# Autodesk Inventor assembly: Zlozenie_glowne
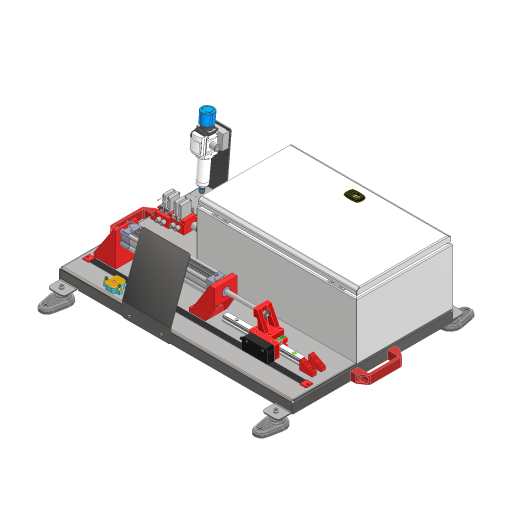
[picture p0: Inventor's stored thumbnail of the model, 512x512]
Saved by Autodesk Inventor 2024.3 (Build 283343000, 343)
## iProperties
Created: 2025-06-06
Part Number: Zlozenie_glowne
Document SubType Name: Assembly
Designer: PM
Author: PM
## Documents named in this file (45)
- C:\MPA - shortPath\magisterka\V3\Workspace\Zlozenie_glowne.iam
- C:\MPA - shortPath\magisterka\V3\Workspace\Stół.iam
- C:\MPA - shortPath\magisterka\V3\Workspace\Zakupowe\hiwin\HGH20CA1R250Z0H_FILE_1\HGH20CA1R250Z0H_FILE_1\HGH20CA1R250Z0H_FILE_1.iam
- C:\MPA - shortPath\magisterka\V3\Workspace\Part1.ipt
- C:\MPA - shortPath\magisterka\V3\Workspace\Zakupowe\silownik_metlawork\AIS2024\1213320200CP-0-0-0--(200_00).iam
- C:\MPA - shortPath\magisterka\V3\Workspace\cc\en-US\DIN 934\DIN 934 - M10 x 1,25.ipt
- C:\MPA - shortPath\magisterka\V3\Workspace\Part6.ipt
- C:\MPA - shortPath\magisterka\V3\Workspace\cc\en-US\DIN 125-1  A\DIN 125 - A 6,4.ipt
- C:\MPA - shortPath\magisterka\V3\Workspace\cc\en-US\DIN 912\DIN 912 - M6 x 1 x 20 x 17,5.ipt
- C:\MPA - shortPath\magisterka\V3\Workspace\cc\en-US\DIN 912\DIN 912 - M6 x 1 x 25 x 22,5.ipt
- C:\MPA - shortPath\magisterka\V3\Workspace\cc\en-US\DIN 934\DIN 934 - M6 x 1.ipt
- C:\MPA - shortPath\magisterka\V3\Workspace\fin.ipt
- C:\MPA - shortPath\magisterka\V3\Workspace\cc\en-US\DIN 912\DIN 912 - M5 x 0,8 x 20 x 18.ipt
- C:\MPA - shortPath\magisterka\V3\Workspace\cc\en-US\DIN 125-1  A\DIN 125 - A 5,3.ipt
- C:\MPA - shortPath\magisterka\V3\Workspace\cc\en-US\DIN 934\DIN 934 - M5 x 0,8.ipt
- C:\MPA - shortPath\magisterka\V3\Workspace\Zakupowe\lika\LIKA SMAX-MB-PRG-L2\LIKA SMAX-MB-PRG-L2\LIKA SMAX-MB-PRG-L2.ipt
- C:\MPA - shortPath\magisterka\V3\Workspace\Zakupowe\lika\MTAZ-500-50-1.ipt
- C:\MPA - shortPath\magisterka\V3\Workspace\Zakupowe\lika\LIKA LKM-1439.ipt
- C:\MPA - shortPath\magisterka\V3\Workspace\cc\en-US\ISO 10642(2)\ISO 10642  - M3  x  10.ipt
- C:\MPA - shortPath\magisterka\V3\Workspace\cc\en-US\DIN 125-1  A\DIN 125 - A 3,2.ipt
- C:\MPA - shortPath\magisterka\V3\Workspace\cc\en-US\DIN 934\DIN 934 - M3 x 0,5.ipt
- C:\MPA - shortPath\magisterka\V3\Workspace\blokada_hiwin.ipt
- C:\MPA - shortPath\magisterka\V3\Workspace\cc\en-US\DIN 912\DIN 912 - M4 x 0,7 x 16 x 14,25.ipt
- C:\MPA - shortPath\magisterka\V3\Workspace\cc\en-US\DIN 125-1  A\DIN 125 - A 4,3.ipt
- C:\MPA - shortPath\magisterka\V3\Workspace\cc\en-US\DIN 934\DIN 934 - M4 x 0,7.ipt
- C:\MPA - shortPath\magisterka\V3\Workspace\Zlozenie_smc.iam
- C:\MPA - shortPath\magisterka\V3\Workspace\Zakupowe\FESTO\MS4-EM1FR-14-D6-E-P-M-AG-MPA-WPE-B\8098374 MS4-EM1FR-1_4-D6-E-P-M-AG-MPA-WPE-B.iam
- C:\MPA - shortPath\magisterka\V3\Workspace\Zakupowe\smc\KQ2S06-01AS_(A) Brass.ipt
- C:\MPA - shortPath\magisterka\V3\Workspace\Part15.ipt
- C:\MPA - shortPath\magisterka\V3\Workspace\cc\en-US\DIN 912\DIN 912 - M4 x 0,7 x 30 x 20.ipt
- C:\MPA - shortPath\magisterka\V3\Workspace\Zakupowe\schneider\NSYS3D5320P_3D-Simplified\NSYS3D5320P_3D-Simplified\NSYS3D5320P_3D-Simplified.iam
- C:\MPA - shortPath\magisterka\V3\Workspace\Uchwyt_ZPP.ipt
- C:\MPA - shortPath\magisterka\V3\Workspace\cc\en-US\Copy of DIN 912 - replaced by DIN EN ISO 4762\Copy of DIN 912 - M5 x 0,8 x 16 x 14.ipt
- C:\MPA - shortPath\magisterka\V3\Workspace\cc\en-US\Copy of DIN 912 - replaced by DIN EN ISO 4762\Copy of DIN 912 - M4 x 0,7 x 20 x 18,25.ipt
- C:\MPA - shortPath\magisterka\V3\Workspace\Zakupowe\elesa\M_443_140-6-CH-C6\M_443_140-6-CH-C6\M_443_140-6-CH-C6.ipt
- C:\MPA - shortPath\magisterka\V3\Workspace\cc\en-US\Copy of DIN 912 - replaced by DIN EN ISO 4762\Copy of DIN 912 - M6 x 1 x 20 x 17,5.ipt
- C:\MPA - shortPath\magisterka\V3\Workspace\cc\en-US\DIN 9021\DIN 9021 - 8,4.ipt
- C:\MPA - shortPath\magisterka\V3\Workspace\cc\en-US\DIN 125-1  A\DIN 125 - A 8,4.ipt
- C:\MPA - shortPath\magisterka\V3\Workspace\cc\en-US\Copy of DIN 912 - replaced by DIN EN ISO 4762\Copy of DIN 912 - M8 x 1,25 x 20 x 16,875.ipt
- C:\MPA - shortPath\magisterka\V3\Workspace\cc\en-US\DIN 934\DIN 934 - M8 x 1,25.ipt
- C:\MPA - shortPath\magisterka\V3\Workspace\Arduino_zlozenie.iam
- C:\MPA - shortPath\magisterka\V3\Workspace\MontazWszafie\Uchwyt_konwerter.iam
- C:\MPA - shortPath\magisterka\V3\Workspace\cc\en-US\Copy of DIN 912 - replaced by DIN EN ISO 4762\Copy of DIN 912 - M4 x 0,7 x 12 x 10,25.ipt
- C:\MPA - shortPath\magisterka\V3\Workspace\PrzyciskSTOP.iam
- C:\MPA - shortPath\magisterka\V3\Workspace\cc\en-US\Copy of DIN 912 - replaced by DIN EN ISO 4762\Copy of DIN 912 - M4 x 0,7 x 25 x 23,25.ipt
## Components (187 placed, 44 different names)
1. Stół:1 [sub-assembly] — Flush:1, Flush:2, Flush:3, Insert:1, Mate:1, Flush:4, Mate:12, Mate:14, Mate:16, Mate:18, Mate:20, Mate:21, Mate:22, Mate:23, Mate:24, Mate:25, Mate:26, Mate:27, Mate:29, Mate:31, Mate:33, Mate:35, Mate:37, Mate:38, Mate:39, Mate:40, Mate:41, Mate:42, Mate:43, Mate:44, Mate:46, Flush:7, Mate:54, Mate:57, Mate:59, Mate:62, Mate:63, Mate:65, Mate:67, Mate:69, Mate:71, Mate:72, Mate:73, Mate:74, Mate:75, Mate:76, Mate:77, Mate:78, Mate:79, Flush:12, Mate:92, Mate:94, Mate:96, Mate:98, Mate:107, Flush:13, Flush:14, Flush:15, Mate:109, Flush:16, Flush:17, Mate:119, Mate:121, Mate:123, Mate:125, Mate:131, Mate:133, Mate:134, Flush:18, Flush:19, Mate:140, Mate:142, Flush:20, Mate:143, Mate:144, Mate:145, Mate:146, Mate:148, Mate:150, Mate:151, Mate:152, Mate:153, Mate:154, Mate:156, Mate:158, Mate:159, Mate:160, Mate:161, Mate:162, Mate:164, Mate:166, Mate:168, Mate:170, Mate:171, Mate:172, Mate:173, Mate:174, Mate:175, Mate:176, Mate:177, Mate:196, Flush:24
2. HGH20CA1R250Z0H_FILE_1:1 [sub-assembly] — Insert:1, Mate:1, Insert:2, Mate:2, Mate:30, Mate:32, Mate:34, Mate:36, Mate:58, Flush:8, Mate:60
3. Part1:1 — Insert:2, Mate:2, Insert:3, Insert:4, Angle:1, Insert:22, Mate:45, Mate:61, Mate:99, Mate:101, Mate:103, Mate:104, Mate:105, Mate:106
4. 1213320200CP-0-0-0--(200_00):1 [sub-assembly] — Insert:3, Angle:1, Insert:5, Mate:3, Flush:4, Insert:31, Insert:32, Insert:33
5. Part6:1 — Insert:5, Mate:3, Mate:4, Mate:5, Mate:6, Mate:7, Mate:8, Mate:9, Mate:10, Mate:11, Mate:13, Mate:15, Mate:17, Mate:19
6. fin:1 — Mate:134, Flush:18, Flush:19, Mate:135, Mate:136, Mate:137, Mate:138, Mate:139, Mate:141
7. LIKA SMAX-MB-PRG-L2:1 — Insert:22, Mate:45, Flush:5, Mate:100, Mate:102
8. MTAZ-500-50-1:1 — Mate:46, Flush:5, Mate:47, Mate:48, Mate:49, Mate:50, Mate:51
9. LIKA LKM-1439:1 — Mate:47, Mate:48, Mate:49, Flush:6, Flush:7, Mate:52, Mate:53
10. LIKA LKM-1439:2 — Flush:6, Mate:50, Mate:51, Mate:55, Mate:56
11. blokada_hiwin:1 — Mate:58, Mate:59, Flush:8, Mate:60, Flush:9, Mate:64, Mate:66, Mate:68, Mate:70
12. blokada_hiwin:2 — Mate:61, Flush:9, Mate:62
13. Zlozenie_smc:1 [sub-assembly] — Mate:79, Flush:12, Flush:15, Mate:126, Mate:127, Mate:128, Mate:129, Mate:130, Mate:132, Flush:23
14. 8098374 MS4-EM1FR-1_4-D6-E-P-M-AG-MPA-WPE-B:1 [sub-assembly] — Insert:42, Mate:108
15. KQ2S06-01AS_(A) Brass:1 — Insert:32
16. KQ2S06-01AS_(A) Brass:2 — Insert:31
17. Part15:1 — Insert:33, Mate:83, Mate:84, Mate:85, Mate:86, Mate:87, Mate:88, Mate:89, Mate:90, Mate:91, Mate:93, Mate:95, Mate:97
18. NSYS3D5320P_3D-Simplified:1 [sub-assembly] — Mate:107, Flush:13, Flush:14, Mate:163, Mate:165, Mate:167, Mate:169
19. Uchwyt_ZPP:1 — Insert:42, Mate:108, Mate:109, Flush:16, Flush:17, Mate:110, Mate:111, Mate:112, Mate:113, Mate:114, Mate:115, Mate:116, Mate:117, Mate:118, Mate:120, Mate:122, Mate:124, Mate:178, Mate:179, Mate:180, Mate:181, Mate:182, Mate:183, Mate:184, Mate:185, Mate:186, Mate:187, Mate:188, Mate:189, Mate:190, Mate:191, Mate:192, Mate:193
20. M_443_140-6-CH-C6:1 — Flush:20, Flush:21, Mate:143, Flush:22, Mate:145, Mate:155, Mate:157
21. M_443_140-6-CH-C6:2 — Flush:21, Mate:144, Flush:22, Mate:147, Mate:149
22. Arduino_zlozenie:1 [sub-assembly]
23. Uchwyt_konwerter:1 [sub-assembly]
24. PrzyciskSTOP:1 [sub-assembly] — Mate:196, Flush:24, Mate:197, Mate:198, Mate:199, Mate:200
25. DIN 125-1 A A 4,3:9 — Mate:178, Mate:179, Insert:79
26. Copy of DIN 912 - replaced by DIN EN ISO 4762 M4 x 12:1 — Insert:79
27. DIN 125-1 A A 4,3:10 — Mate:186, Mate:187, Insert:83
28. DIN 934 - replaced by DIN EN 24032/28673/28674 M4:9 — Insert:83
29. DIN 125-1 A A 4,3:11 — Mate:180, Mate:181, Insert:80
30. DIN 125-1 A A 4,3:12 — Mate:182, Mate:183, Insert:81
31. DIN 125-1 A A 4,3:13 — Mate:184, Mate:185, Insert:82
32. Copy of DIN 912 - replaced by DIN EN ISO 4762 M4 x 12:2 — Insert:80
33. Copy of DIN 912 - replaced by DIN EN ISO 4762 M4 x 12:3 — Insert:81
34. Copy of DIN 912 - replaced by DIN EN ISO 4762 M4 x 12:4 — Insert:82
35. DIN 125-1 A A 4,3:14 — Mate:188, Mate:189, Insert:84
36. DIN 125-1 A A 4,3:15 — Mate:190, Mate:191, Insert:85
37. DIN 125-1 A A 4,3:16 — Mate:192, Mate:193, Insert:86
38. DIN 934 - replaced by DIN EN 24032/28673/28674 M4:10 — Insert:84
39. DIN 934 - replaced by DIN EN 24032/28673/28674 M4:11 — Insert:85
40. DIN 934 - replaced by DIN EN 24032/28673/28674 M4:12 — Insert:86
41. DIN 125-1 A A 4,3:17 — Mate:197, Mate:198, Insert:87
42. Copy of DIN 912 - replaced by DIN EN ISO 4762 M4 x 25:1 — Insert:87
43. DIN 125-1 A A 4,3:18 — Mate:199, Mate:200, Insert:88
44. Copy of DIN 912 - replaced by DIN EN ISO 4762 M4 x 25:2 — Insert:88
45. DIN 9021 8,4:1 — Mate:162, Mate:163, Insert:63
46. DIN 125-1 A A 8,4:1 — Insert:63, Insert:67
47. Copy of DIN 912 - replaced by DIN EN ISO 4762 M8 x 20:1 — Insert:67
48. DIN 125-1 A A 8,4:2 — Mate:170, Mate:171, Insert:71
49. DIN 9021 8,4:2 — Insert:71, Insert:75
50. DIN 934 - replaced by DIN EN 24032/28673/28674 M8:1 — Insert:75
51. DIN 9021 8,4:3 — Mate:164, Mate:165, Insert:64
52. DIN 9021 8,4:4 — Mate:166, Mate:167, Insert:65
53. DIN 9021 8,4:5 — Mate:168, Mate:169, Insert:66
54. DIN 125-1 A A 8,4:3 — Insert:64, Insert:68
55. DIN 125-1 A A 8,4:4 — Insert:65, Insert:69
56. DIN 125-1 A A 8,4:5 — Insert:66, Insert:70
57. Copy of DIN 912 - replaced by DIN EN ISO 4762 M8 x 20:2 — Insert:68
58. Copy of DIN 912 - replaced by DIN EN ISO 4762 M8 x 20:3 — Insert:69
59. Copy of DIN 912 - replaced by DIN EN ISO 4762 M8 x 20:4 — Insert:70
60. DIN 125-1 A A 8,4:6 — Mate:172, Mate:173, Insert:72
61. DIN 125-1 A A 8,4:7 — Mate:174, Mate:175, Insert:73
62. DIN 125-1 A A 8,4:8 — Mate:176, Mate:177, Insert:74
63. DIN 9021 8,4:6 — Insert:72, Insert:76
64. DIN 9021 8,4:7 — Insert:73, Insert:77
65. DIN 9021 8,4:8 — Insert:74, Insert:78
66. DIN 934 - replaced by DIN EN 24032/28673/28674 M8:2 — Insert:76
67. DIN 934 - replaced by DIN EN 24032/28673/28674 M8:3 — Insert:77
68. DIN 934 - replaced by DIN EN 24032/28673/28674 M8:4 — Insert:78
69. DIN 125-1 A A 5,3:5 — Mate:110, Mate:111, Insert:43
70. Copy of DIN 912 - replaced by DIN EN ISO 4762 M5 x 16:1 — Insert:43
71. DIN 125-1 A A 5,3:6 — Mate:118, Mate:119, Insert:47
72. DIN 934 - replaced by DIN EN 24032/28673/28674 M5:5 — Insert:47
73. DIN 125-1 A A 5,3:7 — Mate:112, Mate:113, Insert:44
74. DIN 125-1 A A 5,3:8 — Mate:114, Mate:115, Insert:45
75. DIN 125-1 A A 5,3:9 — Mate:116, Mate:117, Insert:46
76. Copy of DIN 912 - replaced by DIN EN ISO 4762 M5 x 16:2 — Insert:44
77. Copy of DIN 912 - replaced by DIN EN ISO 4762 M5 x 16:3 — Insert:45
78. Copy of DIN 912 - replaced by DIN EN ISO 4762 M5 x 16:4 — Insert:46
79. DIN 125-1 A A 5,3:10 — Mate:120, Mate:121, Insert:48
80. DIN 125-1 A A 5,3:11 — Mate:122, Mate:123, Insert:49
81. DIN 125-1 A A 5,3:12 — Mate:124, Mate:125, Insert:50
82. DIN 934 - replaced by DIN EN 24032/28673/28674 M5:6 — Insert:48
83. DIN 934 - replaced by DIN EN 24032/28673/28674 M5:7 — Insert:49
84. DIN 934 - replaced by DIN EN 24032/28673/28674 M5:8 — Insert:50
85. DIN 125-1 A A 4,3:5 — Mate:126, Mate:127, Insert:51
86. Copy of DIN 912 - replaced by DIN EN ISO 4762 M4 x 20:1 — Insert:51
87. DIN 125-1 A A 4,3:6 — Mate:130, Mate:131, Insert:53
88. DIN 934 - replaced by DIN EN 24032/28673/28674 M4:7 — Insert:53
89. DIN 125-1 A A 4,3:7 — Mate:128, Mate:129, Insert:52
90. Copy of DIN 912 - replaced by DIN EN ISO 4762 M4 x 20:2 — Insert:52
91. DIN 125-1 A A 4,3:8 — Mate:132, Mate:133, Insert:54
92. DIN 934 - replaced by DIN EN 24032/28673/28674 M4:8 — Insert:54
93. DIN 125-1 A A 5,3:13 — Mate:135, Mate:136, Insert:55
94. Copy of DIN 912 - replaced by DIN EN ISO 4762 M5 x 16:5 — Insert:55
95. DIN 125-1 A A 5,3:14 — Mate:139, Mate:140, Insert:57
96. DIN 934 - replaced by DIN EN 24032/28673/28674 M5:9 — Insert:57
97. DIN 125-1 A A 5,3:15 — Mate:137, Mate:138, Insert:56
98. Copy of DIN 912 - replaced by DIN EN ISO 4762 M5 x 16:6 — Insert:56
99. DIN 125-1 A A 5,3:16 — Mate:141, Mate:142, Insert:58
100. DIN 934 - replaced by DIN EN 24032/28673/28674 M5:10 — Insert:58
101. Copy of DIN 912 - replaced by DIN EN ISO 4762 M6 x 20:1 — Mate:146, Mate:147
102. DIN 125-1 A A 6,4:21 — Mate:150, Mate:151, Insert:59
103. DIN 934 - replaced by DIN EN 24032/28673/28674 M6:9 — Insert:59
104. Copy of DIN 912 - replaced by DIN EN ISO 4762 M6 x 20:2 — Mate:148, Mate:149
105. DIN 125-1 A A 6,4:22 — Mate:152, Mate:153, Insert:60
106. DIN 934 - replaced by DIN EN 24032/28673/28674 M6:10 — Insert:60
107. Copy of DIN 912 - replaced by DIN EN ISO 4762 M6 x 20:3 — Mate:154, Mate:155
108. DIN 125-1 A A 6,4:23 — Mate:158, Mate:159, Insert:61
109. DIN 934 - replaced by DIN EN 24032/28673/28674 M6:11 — Insert:61
110. Copy of DIN 912 - replaced by DIN EN ISO 4762 M6 x 20:4 — Mate:156, Mate:157
111. DIN 125-1 A A 6,4:24 — Mate:160, Mate:161, Insert:62
112. DIN 934 - replaced by DIN EN 24032/28673/28674 M6:12 — Insert:62
113. DIN 912 - replaced by DIN EN ISO 4762 M4 x 30:1 — Mate:99, Mate:100
114. DIN 934 - replaced by DIN EN 24032/28673/28674 M4:5 — Mate:103, Mate:104
115. DIN 912 - replaced by DIN EN ISO 4762 M4 x 30:2 — Mate:101, Mate:102
116. DIN 934 - replaced by DIN EN 24032/28673/28674 M4:6 — Mate:105, Mate:106
117. DIN 125-1 A A 6,4:13 — Mate:83, Mate:84, Insert:34
118. DIN 912 - replaced by DIN EN ISO 4762 M6 x 25:5 — Insert:34
119. DIN 125-1 A A 6,4:14 — Mate:91, Mate:92, Insert:38
120. DIN 934 - replaced by DIN EN 24032/28673/28674 M6:5 — Insert:38
121. DIN 125-1 A A 6,4:15 — Mate:85, Mate:86, Insert:35
122. DIN 125-1 A A 6,4:16 — Mate:87, Mate:88, Insert:36
123. DIN 125-1 A A 6,4:17 — Mate:89, Mate:90, Insert:37
124. DIN 912 - replaced by DIN EN ISO 4762 M6 x 25:6 — Insert:35
125. DIN 912 - replaced by DIN EN ISO 4762 M6 x 25:7 — Insert:36
126. DIN 912 - replaced by DIN EN ISO 4762 M6 x 25:8 — Insert:37
127. DIN 125-1 A A 6,4:18 — Mate:93, Mate:94, Insert:39
128. DIN 125-1 A A 6,4:19 — Mate:95, Mate:96, Insert:40
129. DIN 125-1 A A 6,4:20 — Mate:97, Mate:98, Insert:41
130. DIN 934 - replaced by DIN EN 24032/28673/28674 M6:6 — Insert:39
131. DIN 934 - replaced by DIN EN 24032/28673/28674 M6:7 — Insert:40
132. DIN 934 - replaced by DIN EN 24032/28673/28674 M6:8 — Insert:41
133. DIN 912 - replaced by DIN EN ISO 4762 M4 x 16:1 — Mate:63, Mate:64
134. DIN 125-1 A A 4,3:1 — Mate:71, Mate:72, Insert:25
135. DIN 934 - replaced by DIN EN 24032/28673/28674 M4:1 — Insert:25
136. DIN 912 - replaced by DIN EN ISO 4762 M4 x 16:2 — Mate:65, Mate:66
137. DIN 912 - replaced by DIN EN ISO 4762 M4 x 16:3 — Mate:67, Mate:68
138. DIN 912 - replaced by DIN EN ISO 4762 M4 x 16:4 — Mate:69, Mate:70
139. DIN 125-1 A A 4,3:2 — Mate:73, Mate:74, Insert:26
140. DIN 125-1 A A 4,3:3 — Mate:75, Mate:76, Insert:27
141. DIN 125-1 A A 4,3:4 — Mate:77, Mate:78, Insert:28
142. DIN 934 - replaced by DIN EN 24032/28673/28674 M4:2 — Insert:26
143. DIN 934 - replaced by DIN EN 24032/28673/28674 M4:3 — Insert:27
144. DIN 934 - replaced by DIN EN 24032/28673/28674 M4:4 — Insert:28
145. DIN EN ISO 10642 M3  x  10:1 — Mate:52
146. DIN 125-1 A A 3,2:1 — Mate:53, Mate:54, Insert:23
147. DIN 934 - replaced by DIN EN 24032/28673/28674 M3:1 — Insert:23
148. DIN EN ISO 10642 M3  x  10:2 — Mate:55
149. DIN 125-1 A A 3,2:2 — Mate:56, Mate:57, Insert:24
150. DIN 934 - replaced by DIN EN 24032/28673/28674 M3:2 — Insert:24
151. DIN 912 - replaced by DIN EN ISO 4762 M5 x 20:1 — Mate:29, Mate:30
152. DIN 125-1 A A 5,3:1 — Mate:37, Mate:38, Insert:18
153. DIN 934 - replaced by DIN EN 24032/28673/28674 M5:1 — Insert:18
154. DIN 912 - replaced by DIN EN ISO 4762 M5 x 20:2 — Mate:31, Mate:32
155. DIN 912 - replaced by DIN EN ISO 4762 M5 x 20:3 — Mate:33, Mate:34
156. DIN 912 - replaced by DIN EN ISO 4762 M5 x 20:4 — Mate:35, Mate:36
157. DIN 125-1 A A 5,3:2 — Mate:39, Mate:40, Insert:19
158. DIN 125-1 A A 5,3:3 — Mate:41, Mate:42, Insert:20
159. DIN 125-1 A A 5,3:4 — Mate:43, Mate:44, Insert:21
160. DIN 934 - replaced by DIN EN 24032/28673/28674 M5:2 — Insert:19
161. DIN 934 - replaced by DIN EN 24032/28673/28674 M5:3 — Insert:20
162. DIN 934 - replaced by DIN EN 24032/28673/28674 M5:4 — Insert:21
163. DIN 125-1 A A 6,4:1 — Mate:4, Mate:5, Insert:6
164. DIN 912 - replaced by DIN EN ISO 4762 M6 x 20:1 — Insert:6
165. DIN 125-1 A A 6,4:2 — Mate:6, Mate:7, Insert:7
166. DIN 125-1 A A 6,4:3 — Mate:8, Mate:9, Insert:8
167. DIN 125-1 A A 6,4:4 — Mate:10, Mate:11, Insert:9
168. DIN 912 - replaced by DIN EN ISO 4762 M6 x 20:2 — Insert:7
169. DIN 912 - replaced by DIN EN ISO 4762 M6 x 20:3 — Insert:8
170. DIN 912 - replaced by DIN EN ISO 4762 M6 x 20:4 — Insert:9
171. DIN 125-1 A A 6,4:5 — Mate:12, Mate:13, Insert:10
172. DIN 912 - replaced by DIN EN ISO 4762 M6 x 25:1 — Insert:10
173. DIN 125-1 A A 6,4:6 — Mate:20, Mate:21, Insert:14
174. DIN 934 - replaced by DIN EN 24032/28673/28674 M6:1 — Insert:14
175. DIN 125-1 A A 6,4:7 — Mate:14, Mate:15, Insert:11
176. DIN 125-1 A A 6,4:8 — Mate:16, Mate:17, Insert:12
177. DIN 125-1 A A 6,4:9 — Mate:18, Mate:19, Insert:13
178. DIN 912 - replaced by DIN EN ISO 4762 M6 x 25:2 — Insert:11
179. DIN 912 - replaced by DIN EN ISO 4762 M6 x 25:3 — Insert:12
180. DIN 912 - replaced by DIN EN ISO 4762 M6 x 25:4 — Insert:13
181. DIN 125-1 A A 6,4:10 — Mate:22, Mate:23, Insert:15
182. DIN 125-1 A A 6,4:11 — Mate:24, Mate:25, Insert:16
183. DIN 125-1 A A 6,4:12 — Mate:26, Mate:27, Insert:17
184. DIN 934 - replaced by DIN EN 24032/28673/28674 M6:2 — Insert:15
185. DIN 934 - replaced by DIN EN 24032/28673/28674 M6:3 — Insert:16
186. DIN 934 - replaced by DIN EN 24032/28673/28674 M6:4 — Insert:17
187. DIN 934 - replaced by DIN EN 24032/28673/28674 M10 x 1,25:1 — Insert:4
## Relationships (304: Mate 195, Insert 86, Flush 22, Angle 1)
- Flush:1: Stół:1
- Flush:2: Stół:1
- Flush:3: Stół:1
- Insert:1: Stół:1 ↔ HGH20CA1R250Z0H_FILE_1:1
- Mate:1: Stół:1 ↔ HGH20CA1R250Z0H_FILE_1:1
- Insert:2: HGH20CA1R250Z0H_FILE_1:1 ↔ Part1:1
- Mate:2: HGH20CA1R250Z0H_FILE_1:1 ↔ Part1:1
- Insert:3: Part1:1 ↔ 1213320200CP-0-0-0--(200_00):1
- Insert:4: Part1:1 ↔ DIN 934 - replaced by DIN EN 24032/28673/28674 M10 x 1,25:1
- Angle:1 (0 deg): Part1:1 ↔ 1213320200CP-0-0-0--(200_00):1
- Insert:5: 1213320200CP-0-0-0--(200_00):1 ↔ Part6:1
- Mate:3: 1213320200CP-0-0-0--(200_00):1 ↔ Part6:1
- Flush:4 (91.5 mm): Stół:1 ↔ 1213320200CP-0-0-0--(200_00):1
- Mate:4: Part6:1 ↔ DIN 125-1 A A 6,4:1
- Mate:5: Part6:1 ↔ DIN 125-1 A A 6,4:1
- Mate:6: Part6:1 ↔ DIN 125-1 A A 6,4:2
- Mate:7: Part6:1 ↔ DIN 125-1 A A 6,4:2
- Mate:8: Part6:1 ↔ DIN 125-1 A A 6,4:3
- Mate:9: Part6:1 ↔ DIN 125-1 A A 6,4:3
- Mate:10: Part6:1 ↔ DIN 125-1 A A 6,4:4
- Mate:11: Part6:1 ↔ DIN 125-1 A A 6,4:4
- Insert:6: DIN 125-1 A A 6,4:1 ↔ DIN 912 - replaced by DIN EN ISO 4762 M6 x 20:1
- Insert:7: DIN 125-1 A A 6,4:2 ↔ DIN 912 - replaced by DIN EN ISO 4762 M6 x 20:2
- Insert:8: DIN 125-1 A A 6,4:3 ↔ DIN 912 - replaced by DIN EN ISO 4762 M6 x 20:3
- Insert:9: DIN 125-1 A A 6,4:4 ↔ DIN 912 - replaced by DIN EN ISO 4762 M6 x 20:4
- Mate:12: Stół:1 ↔ DIN 125-1 A A 6,4:5
- Mate:13: Part6:1 ↔ DIN 125-1 A A 6,4:5
- Mate:14: Stół:1 ↔ DIN 125-1 A A 6,4:7
- Mate:15: Part6:1 ↔ DIN 125-1 A A 6,4:7
- Mate:16: Stół:1 ↔ DIN 125-1 A A 6,4:8
- Mate:17: Part6:1 ↔ DIN 125-1 A A 6,4:8
- Mate:18: Stół:1 ↔ DIN 125-1 A A 6,4:9
- Mate:19: Part6:1 ↔ DIN 125-1 A A 6,4:9
- Insert:10: DIN 125-1 A A 6,4:5 ↔ DIN 912 - replaced by DIN EN ISO 4762 M6 x 25:1
- Insert:11: DIN 125-1 A A 6,4:7 ↔ DIN 912 - replaced by DIN EN ISO 4762 M6 x 25:2
- Insert:12: DIN 125-1 A A 6,4:8 ↔ DIN 912 - replaced by DIN EN ISO 4762 M6 x 25:3
- Insert:13: DIN 125-1 A A 6,4:9 ↔ DIN 912 - replaced by DIN EN ISO 4762 M6 x 25:4
- Mate:20: Stół:1 ↔ DIN 125-1 A A 6,4:6
- Mate:21: Stół:1 ↔ DIN 125-1 A A 6,4:6
- Mate:22: Stół:1 ↔ DIN 125-1 A A 6,4:10
- Mate:23: Stół:1 ↔ DIN 125-1 A A 6,4:10
- Mate:24: Stół:1 ↔ DIN 125-1 A A 6,4:11
- Mate:25: Stół:1 ↔ DIN 125-1 A A 6,4:11
- Mate:26: Stół:1 ↔ DIN 125-1 A A 6,4:12
- Mate:27: Stół:1 ↔ DIN 125-1 A A 6,4:12
- Insert:14: DIN 125-1 A A 6,4:6 ↔ DIN 934 - replaced by DIN EN 24032/28673/28674 M6:1
- Insert:15: DIN 125-1 A A 6,4:10 ↔ DIN 934 - replaced by DIN EN 24032/28673/28674 M6:2
- Insert:16: DIN 125-1 A A 6,4:11 ↔ DIN 934 - replaced by DIN EN 24032/28673/28674 M6:3
- Insert:17: DIN 125-1 A A 6,4:12 ↔ DIN 934 - replaced by DIN EN 24032/28673/28674 M6:4
- Mate:29: Stół:1 ↔ DIN 912 - replaced by DIN EN ISO 4762 M5 x 20:1
- Mate:30: HGH20CA1R250Z0H_FILE_1:1 ↔ DIN 912 - replaced by DIN EN ISO 4762 M5 x 20:1
- Mate:31: Stół:1 ↔ DIN 912 - replaced by DIN EN ISO 4762 M5 x 20:2
- Mate:32: HGH20CA1R250Z0H_FILE_1:1 ↔ DIN 912 - replaced by DIN EN ISO 4762 M5 x 20:2
- Mate:33: Stół:1 ↔ DIN 912 - replaced by DIN EN ISO 4762 M5 x 20:3
- Mate:34: HGH20CA1R250Z0H_FILE_1:1 ↔ DIN 912 - replaced by DIN EN ISO 4762 M5 x 20:3
- Mate:35: Stół:1 ↔ DIN 912 - replaced by DIN EN ISO 4762 M5 x 20:4
- Mate:36: HGH20CA1R250Z0H_FILE_1:1 ↔ DIN 912 - replaced by DIN EN ISO 4762 M5 x 20:4
- Mate:37: Stół:1 ↔ DIN 125-1 A A 5,3:1
- Mate:38: Stół:1 ↔ DIN 125-1 A A 5,3:1
- Mate:39: Stół:1 ↔ DIN 125-1 A A 5,3:2
- Mate:40: Stół:1 ↔ DIN 125-1 A A 5,3:2
- Mate:41: Stół:1 ↔ DIN 125-1 A A 5,3:3
- Mate:42: Stół:1 ↔ DIN 125-1 A A 5,3:3
- Mate:43: Stół:1 ↔ DIN 125-1 A A 5,3:4
- Mate:44: Stół:1 ↔ DIN 125-1 A A 5,3:4
- Insert:18: DIN 125-1 A A 5,3:1 ↔ DIN 934 - replaced by DIN EN 24032/28673/28674 M5:1
- Insert:19: DIN 125-1 A A 5,3:2 ↔ DIN 934 - replaced by DIN EN 24032/28673/28674 M5:2
- Insert:20: DIN 125-1 A A 5,3:3 ↔ DIN 934 - replaced by DIN EN 24032/28673/28674 M5:3
- Insert:21: DIN 125-1 A A 5,3:4 ↔ DIN 934 - replaced by DIN EN 24032/28673/28674 M5:4
- Insert:22: Part1:1 ↔ LIKA SMAX-MB-PRG-L2:1
- Mate:45: Part1:1 ↔ LIKA SMAX-MB-PRG-L2:1
- Mate:46: Stół:1 ↔ MTAZ-500-50-1:1
- Flush:5 (1 mm): LIKA SMAX-MB-PRG-L2:1 ↔ MTAZ-500-50-1:1
- Mate:47: MTAZ-500-50-1:1 ↔ LIKA LKM-1439:1
- Mate:48: MTAZ-500-50-1:1 ↔ LIKA LKM-1439:1
- Mate:49 (0.1 mm): MTAZ-500-50-1:1 ↔ LIKA LKM-1439:1
- Flush:6: LIKA LKM-1439:1 ↔ LIKA LKM-1439:2
- Mate:50: MTAZ-500-50-1:1 ↔ LIKA LKM-1439:2
- Mate:51: MTAZ-500-50-1:1 ↔ LIKA LKM-1439:2
- Flush:7 (15 mm): Stół:1 ↔ LIKA LKM-1439:1
- Mate:52: LIKA LKM-1439:1 ↔ DIN EN ISO 10642 M3  x  10:1
- Mate:53: LIKA LKM-1439:1 ↔ DIN 125-1 A A 3,2:1
- Mate:54: Stół:1 ↔ DIN 125-1 A A 3,2:1
- Insert:23: DIN 125-1 A A 3,2:1 ↔ DIN 934 - replaced by DIN EN 24032/28673/28674 M3:1
- Mate:55: LIKA LKM-1439:2 ↔ DIN EN ISO 10642 M3  x  10:2
- Mate:56: LIKA LKM-1439:2 ↔ DIN 125-1 A A 3,2:2
- Mate:57: Stół:1 ↔ DIN 125-1 A A 3,2:2
- Insert:24: DIN 125-1 A A 3,2:2 ↔ DIN 934 - replaced by DIN EN 24032/28673/28674 M3:2
- Mate:58 (1 mm): HGH20CA1R250Z0H_FILE_1:1 ↔ blokada_hiwin:1
- Mate:59: Stół:1 ↔ blokada_hiwin:1
- Flush:8: HGH20CA1R250Z0H_FILE_1:1 ↔ blokada_hiwin:1
- Mate:60: HGH20CA1R250Z0H_FILE_1:1 ↔ blokada_hiwin:1
- Mate:61 (2 mm): Part1:1 ↔ blokada_hiwin:2
- Flush:9: blokada_hiwin:1 ↔ blokada_hiwin:2
- Mate:62: Stół:1 ↔ blokada_hiwin:2
- Mate:63: Stół:1 ↔ DIN 912 - replaced by DIN EN ISO 4762 M4 x 16:1
- Mate:64: blokada_hiwin:1 ↔ DIN 912 - replaced by DIN EN ISO 4762 M4 x 16:1
- Mate:65: Stół:1 ↔ DIN 912 - replaced by DIN EN ISO 4762 M4 x 16:2
- Mate:66: blokada_hiwin:1 ↔ DIN 912 - replaced by DIN EN ISO 4762 M4 x 16:2
- Mate:67: Stół:1 ↔ DIN 912 - replaced by DIN EN ISO 4762 M4 x 16:3
- Mate:68: blokada_hiwin:1 ↔ DIN 912 - replaced by DIN EN ISO 4762 M4 x 16:3
- Mate:69: Stół:1 ↔ DIN 912 - replaced by DIN EN ISO 4762 M4 x 16:4
- Mate:70: blokada_hiwin:1 ↔ DIN 912 - replaced by DIN EN ISO 4762 M4 x 16:4
- Mate:71: Stół:1 ↔ DIN 125-1 A A 4,3:1
- Mate:72: Stół:1 ↔ DIN 125-1 A A 4,3:1
- Mate:73: Stół:1 ↔ DIN 125-1 A A 4,3:2
- Mate:74: Stół:1 ↔ DIN 125-1 A A 4,3:2
- Mate:75: Stół:1 ↔ DIN 125-1 A A 4,3:3
- Mate:76: Stół:1 ↔ DIN 125-1 A A 4,3:3
- Mate:77: Stół:1 ↔ DIN 125-1 A A 4,3:4
- Mate:78: Stół:1 ↔ DIN 125-1 A A 4,3:4
- Insert:25: DIN 125-1 A A 4,3:1 ↔ DIN 934 - replaced by DIN EN 24032/28673/28674 M4:1
- Insert:26: DIN 125-1 A A 4,3:2 ↔ DIN 934 - replaced by DIN EN 24032/28673/28674 M4:2
- Insert:27: DIN 125-1 A A 4,3:3 ↔ DIN 934 - replaced by DIN EN 24032/28673/28674 M4:3
- Insert:28: DIN 125-1 A A 4,3:4 ↔ DIN 934 - replaced by DIN EN 24032/28673/28674 M4:4
- Mate:79: Stół:1 ↔ Zlozenie_smc:1
- Flush:12 (179.1 mm): Stół:1 ↔ Zlozenie_smc:1
- Insert:31: 1213320200CP-0-0-0--(200_00):1 ↔ KQ2S06-01AS_(A) Brass:2
- Insert:32: 1213320200CP-0-0-0--(200_00):1 ↔ KQ2S06-01AS_(A) Brass:1
- Insert:33: 1213320200CP-0-0-0--(200_00):1 ↔ Part15:1
- Mate:83: Part15:1 ↔ DIN 125-1 A A 6,4:13
- Mate:84: Part15:1 ↔ DIN 125-1 A A 6,4:13
- Mate:85: Part15:1 ↔ DIN 125-1 A A 6,4:15
- Mate:86: Part15:1 ↔ DIN 125-1 A A 6,4:15
- Mate:87: Part15:1 ↔ DIN 125-1 A A 6,4:16
- Mate:88: Part15:1 ↔ DIN 125-1 A A 6,4:16
- Mate:89: Part15:1 ↔ DIN 125-1 A A 6,4:17
- Mate:90: Part15:1 ↔ DIN 125-1 A A 6,4:17
- Insert:34: DIN 125-1 A A 6,4:13 ↔ DIN 912 - replaced by DIN EN ISO 4762 M6 x 25:5
- Insert:35: DIN 125-1 A A 6,4:15 ↔ DIN 912 - replaced by DIN EN ISO 4762 M6 x 25:6
- Insert:36: DIN 125-1 A A 6,4:16 ↔ DIN 912 - replaced by DIN EN ISO 4762 M6 x 25:7
- Insert:37: DIN 125-1 A A 6,4:17 ↔ DIN 912 - replaced by DIN EN ISO 4762 M6 x 25:8
- Mate:91: Part15:1 ↔ DIN 125-1 A A 6,4:14
- Mate:92: Stół:1 ↔ DIN 125-1 A A 6,4:14
- Mate:93: Part15:1 ↔ DIN 125-1 A A 6,4:18
- Mate:94: Stół:1 ↔ DIN 125-1 A A 6,4:18
- Mate:95: Part15:1 ↔ DIN 125-1 A A 6,4:19
- Mate:96: Stół:1 ↔ DIN 125-1 A A 6,4:19
- Mate:97: Part15:1 ↔ DIN 125-1 A A 6,4:20
- Mate:98: Stół:1 ↔ DIN 125-1 A A 6,4:20
- Insert:38: DIN 125-1 A A 6,4:14 ↔ DIN 934 - replaced by DIN EN 24032/28673/28674 M6:5
- Insert:39: DIN 125-1 A A 6,4:18 ↔ DIN 934 - replaced by DIN EN 24032/28673/28674 M6:6
- Insert:40: DIN 125-1 A A 6,4:19 ↔ DIN 934 - replaced by DIN EN 24032/28673/28674 M6:7
- Insert:41: DIN 125-1 A A 6,4:20 ↔ DIN 934 - replaced by DIN EN 24032/28673/28674 M6:8
- Mate:99: Part1:1 ↔ DIN 912 - replaced by DIN EN ISO 4762 M4 x 30:1
- Mate:100: LIKA SMAX-MB-PRG-L2:1 ↔ DIN 912 - replaced by DIN EN ISO 4762 M4 x 30:1
- Mate:101: Part1:1 ↔ DIN 912 - replaced by DIN EN ISO 4762 M4 x 30:2
- Mate:102: LIKA SMAX-MB-PRG-L2:1 ↔ DIN 912 - replaced by DIN EN ISO 4762 M4 x 30:2
- Mate:103: Part1:1 ↔ DIN 934 - replaced by DIN EN 24032/28673/28674 M4:5
- Mate:104: Part1:1 ↔ DIN 934 - replaced by DIN EN 24032/28673/28674 M4:5
- Mate:105: Part1:1 ↔ DIN 934 - replaced by DIN EN 24032/28673/28674 M4:6
- Mate:106: Part1:1 ↔ DIN 934 - replaced by DIN EN 24032/28673/28674 M4:6
- Mate:107: Stół:1 ↔ NSYS3D5320P_3D-Simplified:1
- Flush:13: Stół:1 ↔ NSYS3D5320P_3D-Simplified:1
- Flush:14: Stół:1 ↔ NSYS3D5320P_3D-Simplified:1
- Flush:15 (12.5 mm): Stół:1 ↔ Zlozenie_smc:1
- Insert:42: 8098374 MS4-EM1FR-1_4-D6-E-P-M-AG-MPA-WPE-B:1 ↔ Uchwyt_ZPP:1
- Mate:108: 8098374 MS4-EM1FR-1_4-D6-E-P-M-AG-MPA-WPE-B:1 ↔ Uchwyt_ZPP:1
- Mate:109: Stół:1 ↔ Uchwyt_ZPP:1
- Flush:16 (6 mm): Stół:1 ↔ Uchwyt_ZPP:1
- Flush:17 (6 mm): Stół:1 ↔ Uchwyt_ZPP:1
- Mate:110: Uchwyt_ZPP:1 ↔ DIN 125-1 A A 5,3:5
- Mate:111: Uchwyt_ZPP:1 ↔ DIN 125-1 A A 5,3:5
- Mate:112: Uchwyt_ZPP:1 ↔ DIN 125-1 A A 5,3:7
- Mate:113: Uchwyt_ZPP:1 ↔ DIN 125-1 A A 5,3:7
- Mate:114: Uchwyt_ZPP:1 ↔ DIN 125-1 A A 5,3:8
- Mate:115: Uchwyt_ZPP:1 ↔ DIN 125-1 A A 5,3:8
- Mate:116: Uchwyt_ZPP:1 ↔ DIN 125-1 A A 5,3:9
- Mate:117: Uchwyt_ZPP:1 ↔ DIN 125-1 A A 5,3:9
- Insert:43: DIN 125-1 A A 5,3:5 ↔ Copy of DIN 912 - replaced by DIN EN ISO 4762 M5 x 16:1
- Insert:44: DIN 125-1 A A 5,3:7 ↔ Copy of DIN 912 - replaced by DIN EN ISO 4762 M5 x 16:2
- Insert:45: DIN 125-1 A A 5,3:8 ↔ Copy of DIN 912 - replaced by DIN EN ISO 4762 M5 x 16:3
- Insert:46: DIN 125-1 A A 5,3:9 ↔ Copy of DIN 912 - replaced by DIN EN ISO 4762 M5 x 16:4
- Mate:118: Uchwyt_ZPP:1 ↔ DIN 125-1 A A 5,3:6
- Mate:119: Stół:1 ↔ DIN 125-1 A A 5,3:6
- Mate:120: Uchwyt_ZPP:1 ↔ DIN 125-1 A A 5,3:10
- Mate:121: Stół:1 ↔ DIN 125-1 A A 5,3:10
- Mate:122: Uchwyt_ZPP:1 ↔ DIN 125-1 A A 5,3:11
- Mate:123: Stół:1 ↔ DIN 125-1 A A 5,3:11
- Mate:124: Uchwyt_ZPP:1 ↔ DIN 125-1 A A 5,3:12
- Mate:125: Stół:1 ↔ DIN 125-1 A A 5,3:12
- Insert:47: DIN 125-1 A A 5,3:6 ↔ DIN 934 - replaced by DIN EN 24032/28673/28674 M5:5
- Insert:48: DIN 125-1 A A 5,3:10 ↔ DIN 934 - replaced by DIN EN 24032/28673/28674 M5:6
- Insert:49: DIN 125-1 A A 5,3:11 ↔ DIN 934 - replaced by DIN EN 24032/28673/28674 M5:7
- Insert:50: DIN 125-1 A A 5,3:12 ↔ DIN 934 - replaced by DIN EN 24032/28673/28674 M5:8
- Mate:126: Zlozenie_smc:1 ↔ DIN 125-1 A A 4,3:5
- Mate:127: Zlozenie_smc:1 ↔ DIN 125-1 A A 4,3:5
- Mate:128: Zlozenie_smc:1 ↔ DIN 125-1 A A 4,3:7
- Mate:129: Zlozenie_smc:1 ↔ DIN 125-1 A A 4,3:7
- Insert:51: DIN 125-1 A A 4,3:5 ↔ Copy of DIN 912 - replaced by DIN EN ISO 4762 M4 x 20:1
- Insert:52: DIN 125-1 A A 4,3:7 ↔ Copy of DIN 912 - replaced by DIN EN ISO 4762 M4 x 20:2
- Mate:130: Zlozenie_smc:1 ↔ DIN 125-1 A A 4,3:6
- Mate:131: Stół:1 ↔ DIN 125-1 A A 4,3:6
- Mate:132: Zlozenie_smc:1 ↔ DIN 125-1 A A 4,3:8
- Mate:133: Stół:1 ↔ DIN 125-1 A A 4,3:8
- Insert:53: DIN 125-1 A A 4,3:6 ↔ DIN 934 - replaced by DIN EN 24032/28673/28674 M4:7
- Insert:54: DIN 125-1 A A 4,3:8 ↔ DIN 934 - replaced by DIN EN 24032/28673/28674 M4:8
- Mate:134: Stół:1 ↔ fin:1
- Flush:18: Stół:1 ↔ fin:1
- Flush:19 (200 mm): Stół:1 ↔ fin:1
- Mate:135: fin:1 ↔ DIN 125-1 A A 5,3:13
- Mate:136: fin:1 ↔ DIN 125-1 A A 5,3:13
- Mate:137: fin:1 ↔ DIN 125-1 A A 5,3:15
- Mate:138: fin:1 ↔ DIN 125-1 A A 5,3:15
- Insert:55: DIN 125-1 A A 5,3:13 ↔ Copy of DIN 912 - replaced by DIN EN ISO 4762 M5 x 16:5
- Insert:56: DIN 125-1 A A 5,3:15 ↔ Copy of DIN 912 - replaced by DIN EN ISO 4762 M5 x 16:6
- Mate:139: fin:1 ↔ DIN 125-1 A A 5,3:14
- Mate:140: Stół:1 ↔ DIN 125-1 A A 5,3:14
- Mate:141: fin:1 ↔ DIN 125-1 A A 5,3:16
- Mate:142: Stół:1 ↔ DIN 125-1 A A 5,3:16
- Insert:57: DIN 125-1 A A 5,3:14 ↔ DIN 934 - replaced by DIN EN 24032/28673/28674 M5:9
- Insert:58: DIN 125-1 A A 5,3:16 ↔ DIN 934 - replaced by DIN EN 24032/28673/28674 M5:10
- Flush:20: Stół:1 ↔ M_443_140-6-CH-C6:1
- Flush:21: M_443_140-6-CH-C6:1 ↔ M_443_140-6-CH-C6:2
- Mate:143: Stół:1 ↔ M_443_140-6-CH-C6:1
- Mate:144: Stół:1 ↔ M_443_140-6-CH-C6:2
- Flush:22: M_443_140-6-CH-C6:1 ↔ M_443_140-6-CH-C6:2
- Mate:145: Stół:1 ↔ M_443_140-6-CH-C6:1
- Mate:146: Stół:1 ↔ Copy of DIN 912 - replaced by DIN EN ISO 4762 M6 x 20:1
- Mate:147: M_443_140-6-CH-C6:2 ↔ Copy of DIN 912 - replaced by DIN EN ISO 4762 M6 x 20:1
- Mate:148: Stół:1 ↔ Copy of DIN 912 - replaced by DIN EN ISO 4762 M6 x 20:2
- Mate:149: M_443_140-6-CH-C6:2 ↔ Copy of DIN 912 - replaced by DIN EN ISO 4762 M6 x 20:2
- Mate:150: Stół:1 ↔ DIN 125-1 A A 6,4:21
- Mate:151: Stół:1 ↔ DIN 125-1 A A 6,4:21
- Mate:152: Stół:1 ↔ DIN 125-1 A A 6,4:22
- Mate:153: Stół:1 ↔ DIN 125-1 A A 6,4:22
- Insert:59: DIN 125-1 A A 6,4:21 ↔ DIN 934 - replaced by DIN EN 24032/28673/28674 M6:9
- Insert:60: DIN 125-1 A A 6,4:22 ↔ DIN 934 - replaced by DIN EN 24032/28673/28674 M6:10
- Mate:154: Stół:1 ↔ Copy of DIN 912 - replaced by DIN EN ISO 4762 M6 x 20:3
- Mate:155: M_443_140-6-CH-C6:1 ↔ Copy of DIN 912 - replaced by DIN EN ISO 4762 M6 x 20:3
- Mate:156: Stół:1 ↔ Copy of DIN 912 - replaced by DIN EN ISO 4762 M6 x 20:4
- Mate:157: M_443_140-6-CH-C6:1 ↔ Copy of DIN 912 - replaced by DIN EN ISO 4762 M6 x 20:4
- Mate:158: Stół:1 ↔ DIN 125-1 A A 6,4:23
- Mate:159: Stół:1 ↔ DIN 125-1 A A 6,4:23
- Mate:160: Stół:1 ↔ DIN 125-1 A A 6,4:24
- Mate:161: Stół:1 ↔ DIN 125-1 A A 6,4:24
- Insert:61: DIN 125-1 A A 6,4:23 ↔ DIN 934 - replaced by DIN EN 24032/28673/28674 M6:11
- Insert:62: DIN 125-1 A A 6,4:24 ↔ DIN 934 - replaced by DIN EN 24032/28673/28674 M6:12
- Mate:162: Stół:1 ↔ DIN 9021 8,4:1
- Mate:163: NSYS3D5320P_3D-Simplified:1 ↔ DIN 9021 8,4:1
- Mate:164: Stół:1 ↔ DIN 9021 8,4:3
- Mate:165: NSYS3D5320P_3D-Simplified:1 ↔ DIN 9021 8,4:3
- Mate:166: Stół:1 ↔ DIN 9021 8,4:4
- Mate:167: NSYS3D5320P_3D-Simplified:1 ↔ DIN 9021 8,4:4
- Mate:168: Stół:1 ↔ DIN 9021 8,4:5
- Mate:169: NSYS3D5320P_3D-Simplified:1 ↔ DIN 9021 8,4:5
- Insert:63: DIN 9021 8,4:1 ↔ DIN 125-1 A A 8,4:1
- Insert:64: DIN 9021 8,4:3 ↔ DIN 125-1 A A 8,4:3
- Insert:65: DIN 9021 8,4:4 ↔ DIN 125-1 A A 8,4:4
- Insert:66: DIN 9021 8,4:5 ↔ DIN 125-1 A A 8,4:5
- Insert:67: DIN 125-1 A A 8,4:1 ↔ Copy of DIN 912 - replaced by DIN EN ISO 4762 M8 x 20:1
- Insert:68: DIN 125-1 A A 8,4:3 ↔ Copy of DIN 912 - replaced by DIN EN ISO 4762 M8 x 20:2
- Insert:69: DIN 125-1 A A 8,4:4 ↔ Copy of DIN 912 - replaced by DIN EN ISO 4762 M8 x 20:3
- Insert:70: DIN 125-1 A A 8,4:5 ↔ Copy of DIN 912 - replaced by DIN EN ISO 4762 M8 x 20:4
- Mate:170: Stół:1 ↔ DIN 125-1 A A 8,4:2
- Mate:171: Stół:1 ↔ DIN 125-1 A A 8,4:2
- Mate:172: Stół:1 ↔ DIN 125-1 A A 8,4:6
- Mate:173: Stół:1 ↔ DIN 125-1 A A 8,4:6
- Mate:174: Stół:1 ↔ DIN 125-1 A A 8,4:7
- Mate:175: Stół:1 ↔ DIN 125-1 A A 8,4:7
- Mate:176: Stół:1 ↔ DIN 125-1 A A 8,4:8
- Mate:177: Stół:1 ↔ DIN 125-1 A A 8,4:8
- Insert:71: DIN 125-1 A A 8,4:2 ↔ DIN 9021 8,4:2
- Insert:72: DIN 125-1 A A 8,4:6 ↔ DIN 9021 8,4:6
- Insert:73: DIN 125-1 A A 8,4:7 ↔ DIN 9021 8,4:7
- Insert:74: DIN 125-1 A A 8,4:8 ↔ DIN 9021 8,4:8
- Insert:75: DIN 9021 8,4:2 ↔ DIN 934 - replaced by DIN EN 24032/28673/28674 M8:1
- Insert:76: DIN 9021 8,4:6 ↔ DIN 934 - replaced by DIN EN 24032/28673/28674 M8:2
- Insert:77: DIN 9021 8,4:7 ↔ DIN 934 - replaced by DIN EN 24032/28673/28674 M8:3
- Insert:78: DIN 9021 8,4:8 ↔ DIN 934 - replaced by DIN EN 24032/28673/28674 M8:4
- Mate:178: Uchwyt_ZPP:1 ↔ DIN 125-1 A A 4,3:9
- Mate:179: Uchwyt_ZPP:1 ↔ DIN 125-1 A A 4,3:9
- Mate:180: Uchwyt_ZPP:1 ↔ DIN 125-1 A A 4,3:11
- Mate:181: Uchwyt_ZPP:1 ↔ DIN 125-1 A A 4,3:11
- Mate:182: Uchwyt_ZPP:1 ↔ DIN 125-1 A A 4,3:12
- Mate:183: Uchwyt_ZPP:1 ↔ DIN 125-1 A A 4,3:12
- Mate:184: Uchwyt_ZPP:1 ↔ DIN 125-1 A A 4,3:13
- Mate:185: Uchwyt_ZPP:1 ↔ DIN 125-1 A A 4,3:13
- Insert:79: DIN 125-1 A A 4,3:9 ↔ Copy of DIN 912 - replaced by DIN EN ISO 4762 M4 x 12:1
- Insert:80: DIN 125-1 A A 4,3:11 ↔ Copy of DIN 912 - replaced by DIN EN ISO 4762 M4 x 12:2
- Insert:81: DIN 125-1 A A 4,3:12 ↔ Copy of DIN 912 - replaced by DIN EN ISO 4762 M4 x 12:3
- Insert:82: DIN 125-1 A A 4,3:13 ↔ Copy of DIN 912 - replaced by DIN EN ISO 4762 M4 x 12:4
- Mate:186: Uchwyt_ZPP:1 ↔ DIN 125-1 A A 4,3:10
- Mate:187: Uchwyt_ZPP:1 ↔ DIN 125-1 A A 4,3:10
- Mate:188: Uchwyt_ZPP:1 ↔ DIN 125-1 A A 4,3:14
- Mate:189: Uchwyt_ZPP:1 ↔ DIN 125-1 A A 4,3:14
- Mate:190: Uchwyt_ZPP:1 ↔ DIN 125-1 A A 4,3:15
- Mate:191: Uchwyt_ZPP:1 ↔ DIN 125-1 A A 4,3:15
- Mate:192: Uchwyt_ZPP:1 ↔ DIN 125-1 A A 4,3:16
- Mate:193: Uchwyt_ZPP:1 ↔ DIN 125-1 A A 4,3:16
- Insert:83: DIN 125-1 A A 4,3:10 ↔ DIN 934 - replaced by DIN EN 24032/28673/28674 M4:9
- Insert:84: DIN 125-1 A A 4,3:14 ↔ DIN 934 - replaced by DIN EN 24032/28673/28674 M4:10
- Insert:85: DIN 125-1 A A 4,3:15 ↔ DIN 934 - replaced by DIN EN 24032/28673/28674 M4:11
- Insert:86: DIN 125-1 A A 4,3:16 ↔ DIN 934 - replaced by DIN EN 24032/28673/28674 M4:12
- Flush:23 (17.5 mm): Zlozenie_smc:1
- Mate:195
- Mate:196: Stół:1 ↔ PrzyciskSTOP:1
- Flush:24 (10 mm): Stół:1 ↔ PrzyciskSTOP:1
- Mate:197: PrzyciskSTOP:1 ↔ DIN 125-1 A A 4,3:17
- Mate:198: PrzyciskSTOP:1 ↔ DIN 125-1 A A 4,3:17
- Mate:199: PrzyciskSTOP:1 ↔ DIN 125-1 A A 4,3:18
- Mate:200: PrzyciskSTOP:1 ↔ DIN 125-1 A A 4,3:18
- Insert:87: DIN 125-1 A A 4,3:17 ↔ Copy of DIN 912 - replaced by DIN EN ISO 4762 M4 x 25:1
- Insert:88: DIN 125-1 A A 4,3:18 ↔ Copy of DIN 912 - replaced by DIN EN ISO 4762 M4 x 25:2
